# Autodesk Inventor assembly: SampleHolder_Soln
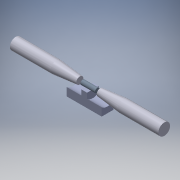
[picture p0: Inventor's stored thumbnail of the model, 180x180]
Saved by Autodesk Inventor 2016 (Build 200138000, 138)
## iProperties
Created: 2017-07-25
Part Number: SampleHolder_Soln
Document SubType Name: Assembly
Designer: bobbyl
Author: bobbyl
## Documents named in this file (4)
- C:\Users\bobbyl\Desktop\CAD QuickStart 2017\Sample_Holder\SampleHolder_Soln.iam
- C:\Users\bobbyl\Desktop\CAD QuickStart 2017\Sample_Holder\Holder_Base.ipt
- C:\Users\bobbyl\Desktop\CAD QuickStart 2017\Sample_Holder\Sample_Material.ipt
- C:\Users\bobbyl\Desktop\CAD QuickStart 2017\Sample_Holder\Compression_Support.ipt
## Components (4 placed, 3 different names)
1. Holder_Base:1 — Mate:1
2. Sample_Material:1 — Mate:1, Mate:2, Mate:3, Mate:4, Mate:5
3. Compression_Support:1 — Mate:2, Mate:3, Symmetry:1
4. Compression_Support:2 — Mate:4, Mate:5, Symmetry:1
## Relationships (6: Mate 5, Symmetry 1)
- Mate:1: Holder_Base:1 ↔ Sample_Material:1
- Mate:2: Sample_Material:1 ↔ Compression_Support:1
- Mate:3 (5 mm): Sample_Material:1 ↔ Compression_Support:1
- Mate:4: Sample_Material:1 ↔ Compression_Support:2
- Mate:5 (5 mm): Sample_Material:1 ↔ Compression_Support:2
- Symmetry:1: Compression_Support:1 ↔ Compression_Support:2
